# Autodesk Inventor assembly: R2_アーム部
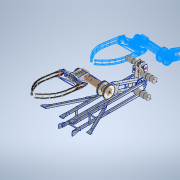
[picture p0: Inventor's stored thumbnail of the model, 180x180]
Saved by Autodesk Inventor 2021 (Build 250183000, 183)
## iProperties
Created: 2022-02-03
Part Number: R2_アーム部
Document SubType Name: Assembly
Designer: hirohumi
Author: hirohumi
## Documents named in this file (13)
- C:\Users\hirohumi\OneDrive\ドキュメント\ロボ研\2022NHKロボコン\R2_version1\R2_アーム部.iam
- C:\Users\hirohumi\OneDrive\ドキュメント\ロボ研\2022NHKロボコン\R2_version1\3軸アームver3\アーム3.iam
- C:\Users\hirohumi\OneDrive\ドキュメント\ロボ研\2022NHKロボコン\R2_version1\オムニ_固定具5.ipt
- C:\Users\hirohumi\OneDrive\ドキュメント\ロボ研\2022NHKロボコン\R2_version1\オムニ_固定具6.ipt
- C:\Users\hirohumi\OneDrive\ドキュメント\ロボ研\2022NHKロボコン\R2_version1\オムニ_角柱8.ipt
- C:\Users\hirohumi\OneDrive\ドキュメント\ロボ研\2022NHKロボコン\R2_version1\3軸アームver2\関節4_側板.ipt
- C:\Users\hirohumi\OneDrive\ドキュメント\ロボ研\2022NHKロボコン\R2_version1\RS-775GM104 v1.ipt
- C:\Users\hirohumi\OneDrive\ドキュメント\ロボ研\2022NHKロボコン\R2_version1\軸_8-80.ipt
- C:\Users\hirohumi\OneDrive\ドキュメント\ロボ研\2022NHKロボコン\R2_version1\オムニ_固定具寸法不明.ipt
- C:\Users\hirohumi\OneDrive\ドキュメント\ロボ研\2022NHKロボコン\R2_version1\オムニ_角柱9.ipt
- C:\Users\hirohumi\OneDrive\ドキュメント\ロボ研\2022NHKロボコン\R2_version1\オムニ_固定具寸法不明2.ipt
- C:\Users\hirohumi\OneDrive\ドキュメント\ロボ研\2022NHKロボコン\R2_version1\オムニ_支え板.ipt
- C:\Users\hirohumi\OneDrive\ドキュメント\ロボ研\2022NHKロボコン\R2_version1\オムニ_支え板横.ipt
## Components (23 placed, 12 different names)
1. アーム3:1 [sub-assembly] — メイト:2, メイト:3
2. オムニ_固定具5:1
3. オムニ_固定具5:2
4. オムニ_固定具6:1
5. オムニ_固定具6:2
6. オムニ_角柱8:1
7. オムニ_角柱8:2
8. オムニ_角柱8:3
9. オムニ_角柱8:4
10. 関節4_側板:1 — メイト:3
11. 関節4_側板:2
12. RS-775GM104 v1:1
13. 軸_8-80:1 — メイト:2
14. オムニ_固定具寸法不明:1
15. オムニ_固定具寸法不明:2
16. オムニ_角柱9:1
17. オムニ_角柱9:2
18. オムニ_固定具寸法不明2:1
19. オムニ_固定具寸法不明2:2
20. オムニ_支え板:1
21. オムニ_支え板:2
22. オムニ_支え板横:1
23. オムニ_支え板横:2
## Relationships (31: Insert 27, Mate 3, Flush 1)
- [Insert]: オムニ_固定具5:2 ↔ オムニ_角柱8:4
- [Insert]: オムニ_固定具5:2 ↔ オムニ_角柱8:4
- [Insert]: オムニ_固定具6:2 ↔ オムニ_角柱8:3
- [Insert]: オムニ_固定具6:2 ↔ オムニ_角柱8:3
- [Insert]: オムニ_固定具6:1 ↔ オムニ_角柱8:2
- [Insert]: オムニ_固定具6:1 ↔ オムニ_角柱8:2
- [Insert]: オムニ_固定具5:1 ↔ オムニ_角柱8:1
- [Insert]: オムニ_固定具5:1 ↔ オムニ_角柱8:1
- [Insert]: オムニ_角柱8:2 ↔ 関節4_側板:1
- [Insert]: オムニ_角柱8:2 ↔ 関節4_側板:1
- [Insert]: オムニ_角柱8:3 ↔ 関節4_側板:2
- [Insert]: オムニ_角柱8:3 ↔ 関節4_側板:2
- [Insert]: 関節4_側板:2 ↔ RS-775GM104 v1:1
- [Mate]: 関節4_側板:2 ↔ RS-775GM104 v1:1
- [Insert]: 関節4_側板:2 ↔ 軸_8-80:1
- [Insert]: オムニ_固定具寸法不明:1 ↔ オムニ_角柱9:1
- [Insert]: オムニ_固定具寸法不明:1 ↔ オムニ_角柱9:1
- [Insert]: オムニ_固定具寸法不明:2 ↔ オムニ_角柱9:2
- [Insert]: オムニ_固定具寸法不明:2 ↔ オムニ_角柱9:2
- [Flush]: オムニ_角柱9:1 ↔ オムニ_固定具寸法不明2:1
- [Insert]: オムニ_角柱8:3 ↔ オムニ_固定具寸法不明2:2
- [Insert]: オムニ_角柱8:3 ↔ オムニ_固定具寸法不明2:2
- [Insert]: オムニ_角柱9:2 ↔ オムニ_固定具寸法不明2:2
- [Insert]: オムニ_角柱8:1 ↔ オムニ_支え板:1
- [Insert]: オムニ_角柱8:4 ↔ オムニ_支え板:1
- [Insert]: オムニ_角柱8:4 ↔ オムニ_支え板:2
- [Insert]: オムニ_角柱8:1 ↔ オムニ_支え板:2
- [Insert]: オムニ_角柱8:4 ↔ オムニ_支え板横:1
- [Insert]: オムニ_角柱8:1 ↔ オムニ_支え板横:2
- メイト:2 [Mate]: アーム3:1 ↔ 軸_8-80:1
- メイト:3 [Mate] (20 mm): アーム3:1 ↔ 関節4_側板:1
